# Autodesk Inventor assembly: Ivot
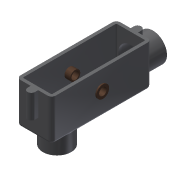
[picture p0: Inventor's stored thumbnail of the model, 180x180]
Saved by Autodesk Inventor 2015 (Build 190159000, 159)
## iProperties
Created: 2015-02-01
Part Number: Ivot
Document SubType Name: Assembly
Designer: Brian
Author: Brian
## Documents named in this file (3)
- C:\Users\Tanner\Documents\GitHub\FIRST-Team-1719-CAD-Team\2015 Robot CAD\Devices\Extender\Pole\Pole.iam
- C:\Users\Tanner\Documents\GitHub\FIRST-Team-1719-CAD-Team\2015 Robot CAD\Devices\Extender\Pole\Access Fitting.ipt
- C:\Users\Tanner\Documents\GitHub\FIRST-Team-1719-CAD-Team\2015 Robot CAD\Devices\Extender\Pole\Flanged Bushing.ipt
## Components (3 placed, 2 different names)
1. Access Fitting:1 — Mate:2, Mate:3, Mate:4
2. Flanged Bushing:1 — Mate:1, Mate:3
3. Flanged Bushing:2 — Mate:1, Mate:2, Mate:4
## Relationships (4: Mate 4)
- Mate:1: Flanged Bushing:1 ↔ Flanged Bushing:2
- Mate:2: Access Fitting:1 ↔ Flanged Bushing:2
- Mate:3: Access Fitting:1 ↔ Flanged Bushing:1
- Mate:4: Access Fitting:1 ↔ Flanged Bushing:2
